# Autodesk Inventor assembly: DD_KVD_004_04
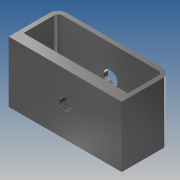
[picture p0: Inventor's stored thumbnail of the model, 180x180]
Saved by Autodesk Inventor 2017.3 (Build 213256000, 256)
## iProperties
Created: 2023-12-15
Part Number: DD_KVD_004_04
Document SubType Name: Weldment
Designer: Darena
Weld Material: Nerezová ocel, kartáčovaná
Author: Darena
## Documents named in this file (3)
- D:\2_Darena\1_Soukrome\02_Inventor soukromé\Dílna RAKO3\Záhora\Pivovar KONTEJNER\S výklopným dnem\DD_KVD_001\DD_KVD_004_04.iam
- D:\2_Darena\1_Soukrome\02_Inventor soukromé\Dílna RAKO3\Záhora\Pivovar KONTEJNER\S výklopným dnem\DD_KVD_001\DD_KVD_004_04_A.ipt
- D:\2_Darena\1_Soukrome\02_Inventor soukromé\Dílna RAKO3\Záhora\Pivovar KONTEJNER\S výklopným dnem\DD_KVD_001\DD_KVD_004_04_B.ipt
## Components (2 placed, 2 different names)
1. DD_KVD_004_04_A:1 — Proti sobě:1, Stejný směr:1, Stejný směr:2
2. DD_KVD_004_04_B:1 — Proti sobě:1, Stejný směr:1, Stejný směr:2
## Relationships (3: Flush 2, Mate 1)
- Proti sobě:1 [Mate]: DD_KVD_004_04_A:1 ↔ DD_KVD_004_04_B:1
- Stejný směr:1 [Flush]: DD_KVD_004_04_A:1 ↔ DD_KVD_004_04_B:1
- Stejný směr:2 [Flush]: DD_KVD_004_04_A:1 ↔ DD_KVD_004_04_B:1
